# Autodesk Inventor assembly: Сборка1
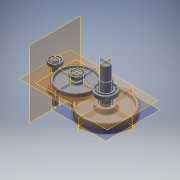
[picture p0: Inventor's stored thumbnail of the model, 180x180]
Saved by Autodesk Inventor 2018 (Build 220112000, 112)
## iProperties
Created: 2018-03-25
Part Number: Сборка1
Material: Типовые
Document SubType Name: Assembly
Designer: kriku
Mass: 4125.82 g
Surface Area: 4507.03 cm^2
Volume: 2397.95 cm^3
Density: 1.72056 g/cm^3
Author: kriku
## Documents named in this file (8)
- C:\Users\kriku\OneDrive\Рабочий стол\6 семестр\курсач ДМ\Куча инви\Сборка1.iam
- C:\Users\kriku\OneDrive\Рабочий стол\6 семестр\курсач ДМ\Куча инви\Вал быстроходный.ipt
- C:\Users\kriku\OneDrive\Рабочий стол\6 семестр\курсач ДМ\Куча инви\Колесо быстроходное.ipt
- C:\Users\kriku\OneDrive\Рабочий стол\6 семестр\курсач ДМ\Куча инви\Вал переходный.ipt
- C:\Users\kriku\OneDrive\Рабочий стол\6 семестр\курсач ДМ\Куча инви\Колесл тихоходное.ipt
- C:\Users\kriku\OneDrive\Рабочий стол\6 семестр\курсач ДМ\Куча инви\Вал тихоходный.ipt
- C:\Users\kriku\OneDrive\Документы\Inventor\Content Center Files\R2018\ru-RU\GOST 8338-75\Подшипник 206 ГОСТ 8338-75.ipt
- C:\Users\kriku\OneDrive\Документы\Inventor\Content Center Files\R2018\ru-RU\GOST 8338-75\Подшипник 211 ГОСТ 8338-75.ipt
## Components (11 placed, 7 different names)
1. Вал быстроходный:1 — Совмещение:1, Совмещение:2, Совмещение:11, Совмещение:12, Совмещение:17, Совмещение:20
2. Колесо быстроходное:1 — Заподлицо:1, Совмещение:1, Совмещение:2, Совмещение:3, Совмещение:4, Совмещение:5
3. Вал переходный:1 — Совмещение:3, Совмещение:4, Совмещение:5, Совмещение:6, Совмещение:7, Совмещение:8, Совмещение:13, Совмещение:14, Совмещение:18, Совмещение:23
4. Колесл тихоходное:1 — Совмещение:6, Совмещение:7, Совмещение:8, Совмещение:9, Заподлицо:2, Совмещение:10
5. Вал тихоходный:1 — Совмещение:9, Заподлицо:2, Совмещение:10, Совмещение:15, Совмещение:16, Совмещение:19, Совмещение:22
6. Подшипник ГОСТ 8338-75 206:1 — Совмещение:11, Совмещение:17
7. Подшипник ГОСТ 8338-75 206:2 — Совмещение:12, Совмещение:20
8. Подшипник ГОСТ 8338-75 206:3 — Совмещение:13, Совмещение:18
9. Подшипник ГОСТ 8338-75 206:4 — Совмещение:14, Совмещение:23
10. Подшипник ГОСТ 8338-75 211:1 — Совмещение:15, Совмещение:22
11. Подшипник ГОСТ 8338-75 211:2 — Совмещение:16, Совмещение:19
## Relationships (24: Mate 22, Flush 2)
- Заподлицо:1 [Flush]: Колесо быстроходное:1
- Совмещение:1 [Mate] (110 mm): Вал быстроходный:1 ↔ Колесо быстроходное:1
- Совмещение:2 [Mate]: Вал быстроходный:1 ↔ Колесо быстроходное:1
- Совмещение:3 [Mate]: Колесо быстроходное:1 ↔ Вал переходный:1
- Совмещение:4 [Mate]: Колесо быстроходное:1 ↔ Вал переходный:1
- Совмещение:5 [Mate]: Колесо быстроходное:1 ↔ Вал переходный:1
- Совмещение:6 [Mate]: Вал переходный:1 ↔ Колесл тихоходное:1
- Совмещение:7 [Mate]: Вал переходный:1 ↔ Колесл тихоходное:1
- Совмещение:8 [Mate] (150 mm): Вал переходный:1 ↔ Колесл тихоходное:1
- Совмещение:9 [Mate]: Колесл тихоходное:1 ↔ Вал тихоходный:1
- Заподлицо:2 [Flush]: Колесл тихоходное:1 ↔ Вал тихоходный:1
- Совмещение:10 [Mate] (11 mm): Колесл тихоходное:1 ↔ Вал тихоходный:1
- Совмещение:11 [Mate]: Вал быстроходный:1 ↔ Подшипник ГОСТ 8338-75 206:1
- Совмещение:12 [Mate]: Вал быстроходный:1 ↔ Подшипник ГОСТ 8338-75 206:2
- Совмещение:13 [Mate]: Вал переходный:1 ↔ Подшипник ГОСТ 8338-75 206:3
- Совмещение:14 [Mate]: Вал переходный:1 ↔ Подшипник ГОСТ 8338-75 206:4
- Совмещение:15 [Mate]: Вал тихоходный:1 ↔ Подшипник ГОСТ 8338-75 211:1
- Совмещение:16 [Mate]: Вал тихоходный:1 ↔ Подшипник ГОСТ 8338-75 211:2
- Совмещение:17 [Mate]: Вал быстроходный:1 ↔ Подшипник ГОСТ 8338-75 206:1
- Совмещение:18 [Mate]: Вал переходный:1 ↔ Подшипник ГОСТ 8338-75 206:3
- Совмещение:19 [Mate]: Вал тихоходный:1 ↔ Подшипник ГОСТ 8338-75 211:2
- Совмещение:20 [Mate]: Вал быстроходный:1 ↔ Подшипник ГОСТ 8338-75 206:2
- Совмещение:22 [Mate]: Вал тихоходный:1 ↔ Подшипник ГОСТ 8338-75 211:1
- Совмещение:23 [Mate]: Вал переходный:1 ↔ Подшипник ГОСТ 8338-75 206:4
